# Autodesk Inventor assembly: 2020 Slider
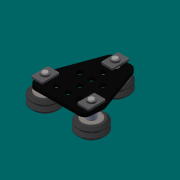
[picture p0: Inventor's stored thumbnail of the model, 180x180]
Saved by Autodesk Inventor 2016 (Build 200138000, 138)
## iProperties
Created: 2015-06-02
Part Number: 2020 Slider
Document SubType Name: Assembly
Designer: Sawaiz Syed
Author: Sawaiz Syed
## Documents named in this file (4)
- C:\Users\Sawaiz\Documents\data\projects\cncBlackBox\yAxis\slider\slider.iam
- C:\Users\Sawaiz\Documents\data\projects\cncBlackBox\yAxis\slider\sliderPlate.ipt
- C:\Users\Sawaiz\Documents\data\projects\cncBlackBox\vWheel\vWheelSpacerTNut.iam
- C:\Users\Sawaiz\Documents\data\projects\cncBlackBox\vWheel\vWheelEccentricTNut.iam
## Components (4 placed, 3 different names)
1. sliderPlate:1 — Mate:1, Mate:2, Mate:3, Mate:4, Angle:3
2. vWheelSpacerTNut:1 [sub-assembly] — Mate:2, Flush:1, Angle:1, Flush:3
3. vWheelEccentricTNut:1 [sub-assembly] — Mate:3, Angle:2, Angle:3, Flush:2, Flush:3
4. vWheelSpacerTNut:2 [sub-assembly] — Mate:1, Flush:1, Mate:4, Angle:1, Angle:2, Flush:2
## Relationships (10: Mate 4, Flush 3, Angle 3)
- Mate:1: sliderPlate:1 ↔ vWheelSpacerTNut:2
- Mate:2: sliderPlate:1 ↔ vWheelSpacerTNut:1
- Mate:3: sliderPlate:1 ↔ vWheelEccentricTNut:1
- Flush:1: vWheelSpacerTNut:1 ↔ vWheelSpacerTNut:2
- Mate:4: sliderPlate:1 ↔ vWheelSpacerTNut:2
- Angle:1 (0 deg): vWheelSpacerTNut:1 ↔ vWheelSpacerTNut:2
- Angle:2 (0 deg): vWheelEccentricTNut:1 ↔ vWheelSpacerTNut:2
- Angle:3 (0 deg): sliderPlate:1 ↔ vWheelEccentricTNut:1
- Flush:2: vWheelEccentricTNut:1 ↔ vWheelSpacerTNut:2
- Flush:3: vWheelSpacerTNut:1 ↔ vWheelEccentricTNut:1
